# Autodesk Inventor assembly: Weapon (Weapon-Side Pulley)
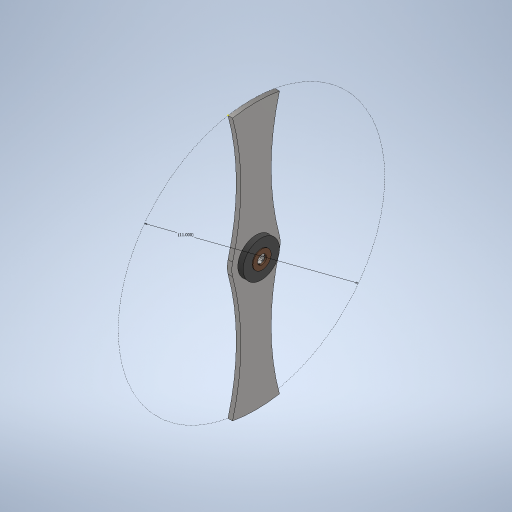
[picture p0: Inventor's stored thumbnail of the model, 512x512]
Saved by Autodesk Inventor 2023.1 (Build 271208000, 208)
## iProperties
Created: 2022-05-08
Part Number: Weapon (Weapon-Side Pulley)
Document SubType Name: Assembly
Designer: NCai2
Mass: 432.97 g
Surface Area: 309.289 cm^2
Volume: 58.6372 cm^3
Density: 7.38387 g/cm^3
Author: NCai2
## Documents named in this file (5)
- E:\Documents\Inventor\0.3rd Lawette - V3.4\Horizontal Weapon Assembly (Type U)\Weapon (Weapon-Side Pulley).iam
- E:\Documents\Inventor\0.3rd Lawette - V3.4\Horizontal Weapon Assembly (Type U)\Blade (Bar 2).ipt
- E:\Documents\Inventor\0.3rd Lawette - V3.4\Horizontal Weapon Assembly (Type U)\7421K2_Ultra-Low-Friction Oil-Embedded Thrust Bearing.ipt
- E:\Documents\Inventor\0.3rd Lawette - V3.4\Horizontal Weapon Assembly (Type U)\5905K497_Needle-Roller Bearing.ipt
- E:\Documents\Inventor\0.3rd Lawette - V3.4\Placeholder (Gear - W).ipt
## Components (5 placed, 4 different names)
1. Blade (Bar 2):1 — Mate:1, Mate:2, Mate:5, Mate:7
2. 7421K2_Ultra-Low-Friction Oil-Embedded Thrust Bearing:1 — Mate:1, Mate:2, Mate:3, Mate:4, Mate:6
3. 7421K2_Ultra-Low-Friction Oil-Embedded Thrust Bearing:2 — Mate:3, Mate:4
4. 5905K497_Needle-Roller Bearing:1 — Mate:5, Mate:6, Mate:8
5. Placeholder (Gear - W):1 — Mate:7, Mate:8
## Relationships (8: Mate 8)
- Mate:1: Blade (Bar 2):1 ↔ 7421K2_Ultra-Low-Friction Oil-Embedded Thrust Bearing:1
- Mate:2: Blade (Bar 2):1 ↔ 7421K2_Ultra-Low-Friction Oil-Embedded Thrust Bearing:1
- Mate:3 (-12.7 mm): 7421K2_Ultra-Low-Friction Oil-Embedded Thrust Bearing:1 ↔ 7421K2_Ultra-Low-Friction Oil-Embedded Thrust Bearing:2
- Mate:4: 7421K2_Ultra-Low-Friction Oil-Embedded Thrust Bearing:1 ↔ 7421K2_Ultra-Low-Friction Oil-Embedded Thrust Bearing:2
- Mate:5: Blade (Bar 2):1 ↔ 5905K497_Needle-Roller Bearing:1
- Mate:6: 7421K2_Ultra-Low-Friction Oil-Embedded Thrust Bearing:1 ↔ 5905K497_Needle-Roller Bearing:1
- Mate:7: Blade (Bar 2):1 ↔ Placeholder (Gear - W):1
- Mate:8: 5905K497_Needle-Roller Bearing:1 ↔ Placeholder (Gear - W):1
